# Autodesk Inventor assembly: Landing_leg_assembly
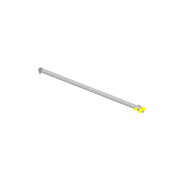
[picture p0: Inventor's stored thumbnail of the model, 180x180]
Saved by Autodesk Inventor 2022 (Build 260153000, 153)
## iProperties
Created: 2022-07-02
Part Number: Landing_leg_assembly
Document SubType Name: Assembly
Designer: dell
Author: dell
## Documents named in this file (5)
- D:\xxxx\Uni\Part IV\MECHENG_700\Part_IV_project_CAD\Bird_skeleton_prototypes\Wing_drone_V1\Landing_leg\Landing_leg_assembly.iam
- D:\xxxx\Uni\Part IV\MECHENG_700\Part_IV_project_CAD\Bird_skeleton_prototypes\Wing_drone_V1\Landing_leg\CF_tube_12mm_500mm.ipt
- D:\xxxx\Uni\Part IV\MECHENG_700\Part_IV_project_CAD\Bird_skeleton_prototypes\Wing_drone_V1\Landing_leg\Landing_leg_clamp_large.ipt
- D:\xxxx\Uni\Part IV\MECHENG_700\Part_IV_project_CAD\Bird_skeleton_prototypes\Wing_drone_V1\Landing_leg\M3_lock_nut.ipt
- D:\xxxx\Uni\Part IV\MECHENG_700\Part_IV_project_CAD\Bird_skeleton_prototypes\Wing_drone_V1\Landing_leg\Landing_leg_clamp_large_shoe.ipt
## Components (5 placed, 4 different names)
1. CF_tube_12mm_500mm:1 — Mate:1, Mate:7, Mate:8, Mate:9
2. Landing_leg_clamp_large:1 — Mate:1, Mate:2, Mate:3, Mate:4, Mate:5, Mate:9
3. M3_lock_nut:1 — Mate:2, Mate:3
4. M3_lock_nut:2 — Mate:4, Mate:5
5. Landing_leg_clamp_large_shoe:1 — Mate:7, Mate:8
## Relationships (8: Mate 8)
- Mate:1: CF_tube_12mm_500mm:1 ↔ Landing_leg_clamp_large:1
- Mate:2: Landing_leg_clamp_large:1 ↔ M3_lock_nut:1
- Mate:3: Landing_leg_clamp_large:1 ↔ M3_lock_nut:1
- Mate:4: Landing_leg_clamp_large:1 ↔ M3_lock_nut:2
- Mate:5: Landing_leg_clamp_large:1 ↔ M3_lock_nut:2
- Mate:7: CF_tube_12mm_500mm:1 ↔ Landing_leg_clamp_large_shoe:1
- Mate:8: CF_tube_12mm_500mm:1 ↔ Landing_leg_clamp_large_shoe:1
- Mate:9: CF_tube_12mm_500mm:1 ↔ Landing_leg_clamp_large:1
